# Autodesk Inventor assembly: Loop Assembly
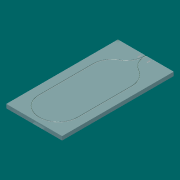
[picture p0: Inventor's stored thumbnail of the model, 180x180]
Saved by Autodesk Inventor 2016 (Build 200138000, 138)
## iProperties
Created: 2015-08-17
Part Number: Loop Assembly
Document SubType Name: Assembly
Designer: Cosmic
Author: Cosmic
## Documents named in this file (4)
- C:\Users\sawaiz\oneDrive\projects\scintillatorPanel\loopLargePanel.iam
- C:\Users\sawaiz\oneDrive\projects\scintillatorPanel\loopLargePanel.ipt
- C:\Users\sawaiz\oneDrive\projects\scintillatorPanel\fiberLargeLoop.ipt
- C:\Users\Sawaiz\OneDrive\projects\scintillatorPanel\Scintillator.xlsx
## Components (2 placed, 2 different names)
1. loopLargePanel:1 — Flush:4, Mate:15, Mate:16
2. fiberLargeLoop:1 — Flush:4, Mate:15, Mate:16
## Relationships (3: Mate 2, Flush 1)
- Flush:4: loopLargePanel:1 ↔ fiberLargeLoop:1
- Mate:15 (0.15 mm): loopLargePanel:1 ↔ fiberLargeLoop:1
- Mate:16 (0.15 mm): loopLargePanel:1 ↔ fiberLargeLoop:1
## Named parameters: OpticalFiberClearence = 0.15 mm, MPPCClearence = 0.075 mm, FiberSensorClerence = 0.5 mm, OpticalFiberDiameter = 1 mm, ScintillatorThickness = 10 mm, SmallTrackDiameter = 175 mm, LargeTrackRatio = 3, ScintillatorEdgeClearence = 3 mm, ScintillatorWidth = 145 mm, ScintillatorHeight = 290 mm, ShallowTrackDepth = 1.3 mm, MPPCSensorClearence = 1.45 mm, MPPCSensorOffsett = 2.105 mm, MPPCWidth = 5.9 mm, MPPCHeight = 6.55 mm, FiberEdgeOffsett = 5 mm, MPPCDepth = 1 mm, LongFiberAngle = 30 deg, ShortFiberAngle = 78 deg, LoopLargeTrackRatio = 1.1, LoopSmallTrackDiameter = 90 mm, MountingScrewDepth = 5 mm, MountingScrewOffsett = 12 mm, LoopLength = 140 mm
